# Autodesk Inventor assembly: Full assembly
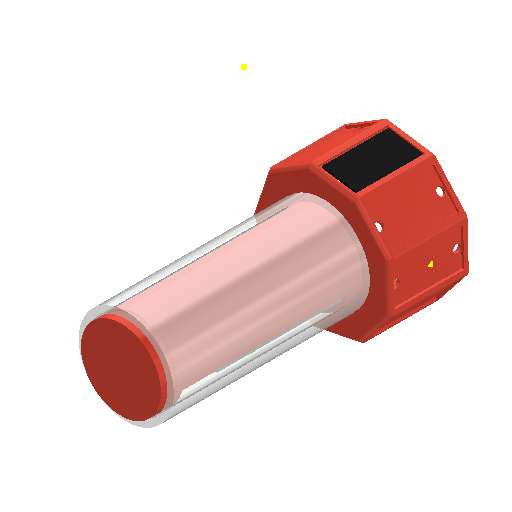
[picture p0: Inventor's stored thumbnail of the model, 512x512]
Saved by Autodesk Inventor 2025 (Build 290162000, 162)
## iProperties
Created: 2025-04-17
Part Number: Full assembly
Document SubType Name: Assembly
Designer: MK92
Sending System: Autodesk Translation Framework v14.4.0.0
Preprocessor: ST-DEVELOPER v20.1
Title: Full assembly.step
## Documents named in this file (7)
- C:\Users\MK92\OneDrive - University of South Carolina\UAV-Deployable-Stage-Height-Sensor\system_design\Georgetown\V0.5\CAD\Inventor files\Full assembly.iam
- C:\Users\MK92\OneDrive - University of South Carolina\UAV-Deployable-Stage-Height-Sensor\system_design\Georgetown\V0.5\CAD\Full assembly\PCB tray CAD v2.ipt
- C:\Users\MK92\OneDrive - University of South Carolina\UAV-Deployable-Stage-Height-Sensor\system_design\Georgetown\V0.5\CAD\Full assembly\Clear Tube v19.iam
- C:\Users\MK92\OneDrive - University of South Carolina\UAV-Deployable-Stage-Height-Sensor\system_design\Georgetown\V0.5\CAD\Full assembly\Battery.ipt
- C:\Users\MK92\OneDrive - University of South Carolina\UAV-Deployable-Stage-Height-Sensor\system_design\Georgetown\V0.5\CAD\Full assembly\main_board v1.iam
- C:\Users\MK92\OneDrive - University of South Carolina\UAV-Deployable-Stage-Height-Sensor\system_design\Georgetown\V0.5\CAD\Ultrasonic HCSR04\Ultrasonic HCSR04.ipt
- C:\Users\MK92\OneDrive - University of South Carolina\UAV-Deployable-Stage-Height-Sensor\system_design\Georgetown\V0.5\CAD\V0.5.2\Solar Panel.ipt
## Components (6 placed, 6 different names)
1. PCB tray CAD v2:1 — Mate:1, Mate:2
2. Clear Tube v19:1 [sub-assembly]
3. Battery:1
4. main_board v1:1 [sub-assembly]
5. Ultrasonic HCSR04:1
6. Solar Panel:1 — Mate:1, Mate:2
## Relationships (2: Mate 2)
- Mate:1: PCB tray CAD v2:1 ↔ Solar Panel:1
- Mate:2 (7.051 mm): PCB tray CAD v2:1 ↔ Solar Panel:1
